# Autodesk Inventor assembly: Enclosure_Base
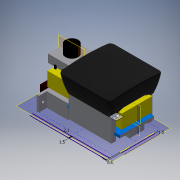
[picture p0: Inventor's stored thumbnail of the model, 180x180]
Saved by Autodesk Inventor 2019.4 (Build 234330000, 330)
## iProperties
Created: 2021-06-28
Part Number: Enclosure_Base
Document SubType Name: Assembly
Designer: keshav
Author: keshav
## Documents named in this file (2)
- D:\Keshav\Maker\Microview_Pendant\Microview_Pendant\CAD\Enclosure_Base.iam
- D:\Keshav\Maker\Microview_Pendant\Microview_Pendant\CAD\Microview_and_Headers.iam
## Components (1 placed, 1 different names)
1. Microview_and_Headers:1 [sub-assembly] — Flush:1
## Relationships (1: Flush 1)
- Flush:1: Microview_and_Headers:1
